# Autodesk Inventor assembly: x reduction assembly 2
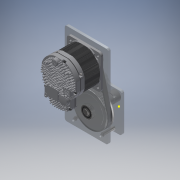
[picture p0: Inventor's stored thumbnail of the model, 180x180]
Saved by Autodesk Inventor 2019 (Build 230136000, 136)
## iProperties
Created: 2018-08-04
Part Number: x reduction assembly 2
Document SubType Name: Assembly
Designer: torba
Author: torba
## Documents named in this file (16)
- C:\Users\torba\OneDrive\Documents\Inventor\Plasma 5x10\x reduction assembly 2.iam
- C:\Users\torba\OneDrive\Documents\Inventor\Plasma 5x10\CPM-341x\CPM-_ _ _ _ - 3411_-LS.ipt
- C:\Users\torba\OneDrive\Documents\Inventor\Plasma 5x10\z gearing adapter.ipt
- C:\Users\torba\OneDrive\Documents\Inventor\Plasma 5x10\PARTserver02018080405093218712503063ca5d5\AIS2018\ATP16XL050-A-PUF.iam
- C:\Users\torba\OneDrive\Documents\Inventor\Plasma 5x10\PARTserver02018080405260113312514063ca5d5\AIS2018\ATP50XL050-A-PUF.iam
- C:\Users\torba\OneDrive\Documents\Inventor\Plasma 5x10\z gearing adapter bottom.ipt
- C:\Users\torba\OneDrive\Documents\Inventor\Plasma 5x10\AST_Bearings_FR8-2RS\AST_Bearings_FR8-2RS.ipt
- C:\Users\torba\OneDrive\Documents\Inventor\Plasma 5x10\idler.ipt
- C:\Users\torba\OneDrive\Documents\Inventor\Plasma 5x10\belt x.ipt
- C:\Users\torba\OneDrive\Documents\Inventor\Plasma 5x10\spacer x.ipt
- C:\Users\torba\OneDrive\Documents\Inventor\Plasma 5x10\PSC1024 Gear (Simplified).ipt
- C:\Users\torba\OneDrive\Documents\Inventor\Plasma 5x10\keyed shaft 80mm.ipt
- C:\Users\torba\OneDrive\Documents\Inventor\Plasma 5x10\spacer x rear.ipt
- C:\Users\torba\OneDrive\Documents\Inventor\Plasma 5x10\x shaft spacer.ipt
- C:\Users\torba\OneDrive\Documents\Inventor\Plasma 5x10\idler spacer.ipt
- C:\Users\torba\OneDrive\Documents\Inventor\Plasma 5x10\shaft washer 1mm.ipt
## Components (17 placed, 15 different names)
1. CPM-_ _ _ _ - 3411_-LS:1
2. z gearing adapter:1 — Mate:29
3. ATP16XL050-A-PUF:1 [sub-assembly]
4. ATP50XL050-A-PUF:1 [sub-assembly] — Mate:26
5. z gearing adapter bottom:1 — Mate:28
6. AST_Bearings_FR8-2RS:1 — Mate:31
7. AST_Bearings_FR8-2RS:2 — Mate:27
8. idler:1 — Mate:30
9. belt x:1
10. spacer x:1
11. spacer x rear:1 — Mate:28
12. spacer x:3
13. PSC1024 Gear (Simplified):1 — Flush:3, Mate:23
14. keyed shaft 80mm:1 — Flush:3, Mate:23, Mate:25, Mate:27, Mate:32
15. x shaft spacer:1 — Mate:25, Mate:26
16. idler spacer:1 — Mate:29, Mate:30
17. shaft washer 1mm:1 — Mate:31, Mate:32
## Relationships (35: Mate 31, Flush 3, Angle 1)
- [Mate]: CPM-_ _ _ _ - 3411_-LS:1 ↔ z gearing adapter:1
- [Mate]: CPM-_ _ _ _ - 3411_-LS:1 ↔ z gearing adapter:1
- [Angle] (270 deg): CPM-_ _ _ _ - 3411_-LS:1 ↔ z gearing adapter:1
- [Mate]: CPM-_ _ _ _ - 3411_-LS:1 ↔ ATP16XL050-A-PUF:1
- [Flush]: ATP16XL050-A-PUF:1 ↔ ATP50XL050-A-PUF:1
- [Mate]: z gearing adapter:1 ↔ ATP50XL050-A-PUF:1
- [Mate]: z gearing adapter bottom:1 ↔ AST_Bearings_FR8-2RS:2
- [Mate]: z gearing adapter bottom:1 ↔ AST_Bearings_FR8-2RS:2
- [Mate] (5 mm): ATP50XL050-A-PUF:1 ↔ AST_Bearings_FR8-2RS:2
- [Mate]: z gearing adapter:1 ↔ AST_Bearings_FR8-2RS:1
- [Mate] (1 mm): ATP50XL050-A-PUF:1 ↔ AST_Bearings_FR8-2RS:1
- [Mate]: z gearing adapter:1 ↔ AST_Bearings_FR8-2RS:1
- [Mate] (4.064 mm): z gearing adapter:1 ↔ idler:1
- [Mate]: z gearing adapter:1 ↔ idler:1
- [Mate] (1 mm): ATP16XL050-A-PUF:1 ↔ belt x:1
- [Mate]: CPM-_ _ _ _ - 3411_-LS:1 ↔ belt x:1
- [Mate]: AST_Bearings_FR8-2RS:2 ↔ belt x:1
- [Mate]: z gearing adapter bottom:1 ↔ spacer x:1
- [Mate]: z gearing adapter bottom:1 ↔ spacer x rear:1
- [Mate]: z gearing adapter bottom:1 ↔ spacer x:3
- [Mate]: z gearing adapter:1 ↔ spacer x rear:1
- [Mate]: z gearing adapter:1 ↔ spacer x:3
- [Mate]: z gearing adapter:1 ↔ spacer x:1
- [Mate]: AST_Bearings_FR8-2RS:1 ↔ PSC1024 Gear (Simplified):1
- [Flush] (35 mm): z gearing adapter bottom:1 ↔ PSC1024 Gear (Simplified):1
- Flush:3 (-2 mm): PSC1024 Gear (Simplified):1 ↔ keyed shaft 80mm:1
- Mate:23: PSC1024 Gear (Simplified):1 ↔ keyed shaft 80mm:1
- Mate:25: keyed shaft 80mm:1 ↔ x shaft spacer:1
- Mate:26: ATP50XL050-A-PUF:1 ↔ x shaft spacer:1
- Mate:27: AST_Bearings_FR8-2RS:2 ↔ keyed shaft 80mm:1
- Mate:28: z gearing adapter bottom:1 ↔ spacer x rear:1
- Mate:29: z gearing adapter:1 ↔ idler spacer:1
- Mate:30: idler:1 ↔ idler spacer:1
- Mate:31: AST_Bearings_FR8-2RS:1 ↔ shaft washer 1mm:1
- Mate:32: keyed shaft 80mm:1 ↔ shaft washer 1mm:1
